# Autodesk Inventor assembly: Wheel Assembly
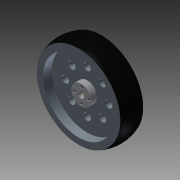
[picture p0: Inventor's stored thumbnail of the model, 180x180]
Saved by Autodesk Inventor 2015 (Build 190159000, 159)
## iProperties
Created: 2015-09-28
Part Number: Wheel Assembly
Document SubType Name: Assembly
Designer: Jing-Chen
Author: Jing-Chen
## Documents named in this file (4)
- C:\Users\Jing-Chen\Desktop\Bionic Hybrids 2016\Bionic-Hybrids\CAD\Drivetrain\Sub-Assemblies\Wheel Assembly.iam
- C:\Users\Jing-Chen\Desktop\Bionic Hybrids 2016\Bionic-Hybrids\Stock\Wheel-Medium(4 in) - 739055.ipt
- C:\Users\Jing-Chen\Desktop\Bionic Hybrids 2016\Bionic-Hybrids\Stock\Shaft Collar-Setscrew, Axle, Mountable - 739079.iam
- C:\Users\Jing-Chen\Desktop\Bionic Hybrids 2016\Bionic-Hybrids\Stock\Screw 0.5in - 739097.ipt
## Components (6 placed, 3 different names)
1. Wheel-Medium(4 in) - 739055:1 — Mate:1, Mate:2, Mate:7, Mate:8, Mate:9, Mate:10
2. Shaft Collar-Setscrew, Axle, Mountable - 739079:1 [sub-assembly] — Mate:1, Mate:2, Mate:3, Mate:4, Mate:5, Mate:6
3. Screw 0.5in - 739097:1 — Mate:3, Mate:10
4. Screw 0.5in - 739097:2 — Mate:4, Mate:8
5. Screw 0.5in - 739097:3 — Mate:5, Mate:7
6. Screw 0.5in - 739097:4 — Mate:6, Mate:9
## Relationships (10: Mate 10)
- Mate:1: Wheel-Medium(4 in) - 739055:1 ↔ Shaft Collar-Setscrew, Axle, Mountable - 739079:1
- Mate:2: Wheel-Medium(4 in) - 739055:1 ↔ Shaft Collar-Setscrew, Axle, Mountable - 739079:1
- Mate:3: Shaft Collar-Setscrew, Axle, Mountable - 739079:1 ↔ Screw 0.5in - 739097:1
- Mate:4: Shaft Collar-Setscrew, Axle, Mountable - 739079:1 ↔ Screw 0.5in - 739097:2
- Mate:5: Shaft Collar-Setscrew, Axle, Mountable - 739079:1 ↔ Screw 0.5in - 739097:3
- Mate:6: Shaft Collar-Setscrew, Axle, Mountable - 739079:1 ↔ Screw 0.5in - 739097:4
- Mate:7: Wheel-Medium(4 in) - 739055:1 ↔ Screw 0.5in - 739097:3
- Mate:8: Wheel-Medium(4 in) - 739055:1 ↔ Screw 0.5in - 739097:2
- Mate:9: Wheel-Medium(4 in) - 739055:1 ↔ Screw 0.5in - 739097:4
- Mate:10: Wheel-Medium(4 in) - 739055:1 ↔ Screw 0.5in - 739097:1
